(part 1 of 3)
# Autodesk Inventor assembly: DesignRootModel^PCB_ESP32-C3-MINI-1_V1(2)_PCB_ESP32-C3-MINI-1_V1
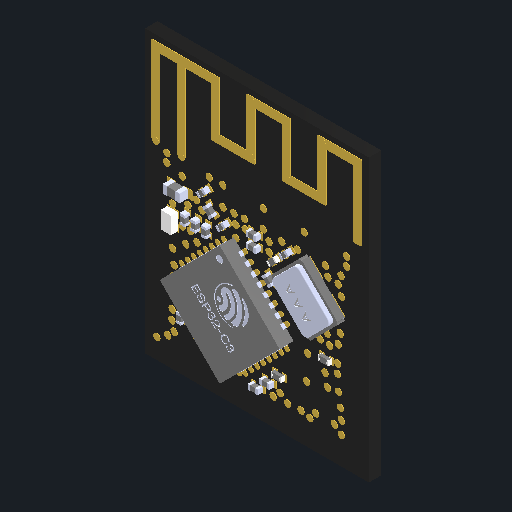
[picture p0: Inventor's stored thumbnail of the model, 512x512]
Saved by Autodesk Inventor 2026.1 (Build 301233000, 233)
## iProperties
Created: 2025-11-22
Part Number: DesignRootModel^PCB_ESP32-C3-MINI-1_V1(2)_PCB_ESP32-C3-MINI-1_V1
Document SubType Name: Assembly
Designer: micyg
Author: micyg
## Documents named in this file (333)
- C:\Users\micyg\Projects\virtual_pet\VirtualBlob\Mechanical\boards\MainBoard\MainBoard_0_4_0\VirtualBlob_MainBoard_0.4.0\VirtualBlob_MainBoard_0.4.0\DesignRootModel^PCB_ESP32-C3-MINI-1_V1(2)_PCB_ESP32-C3-MINI-1_.iam
- C:\Users\micyg\Projects\virtual_pet\VirtualBlob\Mechanical\boards\MainBoard\MainBoard_0_4_0\VirtualBlob_MainBoard_0.4.0\VirtualBlob_MainBoard_0.4.0\Submodel-SOD882_part^DesignRootModel_PCB_ESP32-C3-MINI-1_V1(2).iam
- C:\Users\micyg\Projects\virtual_pet\VirtualBlob\Mechanical\boards\MainBoard\MainBoard_0_4_0\VirtualBlob_MainBoard_0.4.0\VirtualBlob_MainBoard_0.4.0\Submodel-R0201_part^DesignRootModel_PCB_ESP32-C3-MINI-1_V1(2)_.iam
- C:\Users\micyg\Projects\virtual_pet\VirtualBlob\Mechanical\boards\MainBoard\MainBoard_0_4_0\VirtualBlob_MainBoard_0.4.0\VirtualBlob_MainBoard_0.4.0\Submodel-MINI-ANT-TYPED-H_1968823293_part^DesignRootModel_PCB_.iam
- C:\Users\micyg\Projects\virtual_pet\VirtualBlob\Mechanical\boards\MainBoard\MainBoard_0_4_0\VirtualBlob_MainBoard_0.4.0\VirtualBlob_MainBoard_0.4.0\Submodel-C0402_part^DesignRootModel_PCB_ESP32-C3-MINI-1_V1(2)_.iam
- C:\Users\micyg\Projects\virtual_pet\VirtualBlob\Mechanical\boards\MainBoard\MainBoard_0_4_0\VirtualBlob_MainBoard_0.4.0\VirtualBlob_MainBoard_0.4.0\Submodel-R0201_part^DesignRootModel_PCB_ESP32-C3-MINI-1_V1(2)__1.iam
- C:\Users\micyg\Projects\virtual_pet\VirtualBlob\Mechanical\boards\MainBoard\MainBoard_0_4_0\VirtualBlob_MainBoard_0.4.0\VirtualBlob_MainBoard_0.4.0\Submodel-C0201_part^DesignRootModel_PCB_ESP32-C3-MINI-1_V1(2)_.iam
- C:\Users\micyg\Projects\virtual_pet\VirtualBlob\Mechanical\boards\MainBoard\MainBoard_0_4_0\VirtualBlob_MainBoard_0.4.0\VirtualBlob_MainBoard_0.4.0\Submodel-R0201_part^DesignRootModel_PCB_ESP32-C3-MINI-1_V1(2)__2.iam
- C:\Users\micyg\Projects\virtual_pet\VirtualBlob\Mechanical\boards\MainBoard\MainBoard_0_4_0\VirtualBlob_MainBoard_0.4.0\VirtualBlob_MainBoard_0.4.0\Submodel-C0201_part^DesignRootModel_PCB_ESP32-C3-MINI-1_V1(2)__1.iam
- C:\Users\micyg\Projects\virtual_pet\VirtualBlob\Mechanical\boards\MainBoard\MainBoard_0_4_0\VirtualBlob_MainBoard_0.4.0\VirtualBlob_MainBoard_0.4.0\Submodel-C0201_part^DesignRootModel_PCB_ESP32-C3-MINI-1_V1(2)__2.iam
- C:\Users\micyg\Projects\virtual_pet\VirtualBlob\Mechanical\boards\MainBoard\MainBoard_0_4_0\VirtualBlob_MainBoard_0.4.0\VirtualBlob_MainBoard_0.4.0\Submodel-C0201_part^DesignRootModel_PCB_ESP32-C3-MINI-1_V1(2)__3.iam
- C:\Users\micyg\Projects\virtual_pet\VirtualBlob\Mechanical\boards\MainBoard\MainBoard_0_4_0\VirtualBlob_MainBoard_0.4.0\VirtualBlob_MainBoard_0.4.0\Submodel-C0201_part^DesignRootModel_PCB_ESP32-C3-MINI-1_V1(2)__4.iam
- C:\Users\micyg\Projects\virtual_pet\VirtualBlob\Mechanical\boards\MainBoard\MainBoard_0_4_0\VirtualBlob_MainBoard_0.4.0\VirtualBlob_MainBoard_0.4.0\Submodel-C0201_part^DesignRootModel_PCB_ESP32-C3-MINI-1_V1(2)__5.iam
- C:\Users\micyg\Projects\virtual_pet\VirtualBlob\Mechanical\boards\MainBoard\MainBoard_0_4_0\VirtualBlob_MainBoard_0.4.0\VirtualBlob_MainBoard_0.4.0\Submodel-C0201_part^DesignRootModel_PCB_ESP32-C3-MINI-1_V1(2)__6.iam
- C:\Users\micyg\Projects\virtual_pet\VirtualBlob\Mechanical\boards\MainBoard\MainBoard_0_4_0\VirtualBlob_MainBoard_0.4.0\VirtualBlob_MainBoard_0.4.0\Submodel-C0201_part^DesignRootModel_PCB_ESP32-C3-MINI-1_V1(2)__7.iam
- C:\Users\micyg\Projects\virtual_pet\VirtualBlob\Mechanical\boards\MainBoard\MainBoard_0_4_0\VirtualBlob_MainBoard_0.4.0\VirtualBlob_MainBoard_0.4.0\Submodel-C0201_part^DesignRootModel_PCB_ESP32-C3-MINI-1_V1(2)__8.iam
- C:\Users\micyg\Projects\virtual_pet\VirtualBlob\Mechanical\boards\MainBoard\MainBoard_0_4_0\VirtualBlob_MainBoard_0.4.0\VirtualBlob_MainBoard_0.4.0\Submodel-C0201_part^DesignRootModel_PCB_ESP32-C3-MINI-1_V1(2)__9.iam
- C:\Users\micyg\Projects\virtual_pet\VirtualBlob\Mechanical\boards\MainBoard\MainBoard_0_4_0\VirtualBlob_MainBoard_0.4.0\VirtualBlob_MainBoard_0.4.0\Submodel-L0201_part^DesignRootModel_PCB_ESP32-C3-MINI-1_V1(2)_.iam
- C:\Users\micyg\Projects\virtual_pet\VirtualBlob\Mechanical\boards\MainBoard\MainBoard_0_4_0\VirtualBlob_MainBoard_0.4.0\VirtualBlob_MainBoard_0.4.0\Submodel-L0201_part^DesignRootModel_PCB_ESP32-C3-MINI-1_V1(2)__1.iam
- C:\Users\micyg\Projects\virtual_pet\VirtualBlob\Mechanical\boards\MainBoard\MainBoard_0_4_0\VirtualBlob_MainBoard_0.4.0\VirtualBlob_MainBoard_0.4.0\Submodel-XTAL3225_part^DesignRootModel_PCB_ESP32-C3-MINI-1_V1(.iam
- C:\Users\micyg\Projects\virtual_pet\VirtualBlob\Mechanical\boards\MainBoard\MainBoard_0_4_0\VirtualBlob_MainBoard_0.4.0\VirtualBlob_MainBoard_0.4.0\Submodel-QFN32_0P5_5_part^DesignRootModel_PCB_ESP32-C3-MINI-1_.iam
- C:\Users\micyg\Projects\virtual_pet\VirtualBlob\Mechanical\boards\MainBoard\MainBoard_0_4_0\VirtualBlob_MainBoard_0.4.0\VirtualBlob_MainBoard_0.4.0\Submodel-C0201_part^DesignRootModel_PCB_ESP32-C3-MINI-1_V1(2)__10.iam
- C:\Users\micyg\Projects\virtual_pet\VirtualBlob\Mechanical\boards\MainBoard\MainBoard_0_4_0\VirtualBlob_MainBoard_0.4.0\VirtualBlob_MainBoard_0.4.0\uid__4^DesignRootModel_PCB_ESP32-C3-MINI-1_V1(2)_PCB_ESP32-C3-.ipt
- C:\Users\micyg\Projects\virtual_pet\VirtualBlob\Mechanical\boards\MainBoard\MainBoard_0_4_0\VirtualBlob_MainBoard_0.4.0\VirtualBlob_MainBoard_0.4.0\uid__4-22^DesignRootModel_PCB_ESP32-C3-MINI-1_V1(2)_PCB_ESP32-.ipt
- C:\Users\micyg\Projects\virtual_pet\VirtualBlob\Mechanical\boards\MainBoard\MainBoard_0_4_0\VirtualBlob_MainBoard_0.4.0\VirtualBlob_MainBoard_0.4.0\uid__4-23^DesignRootModel_PCB_ESP32-C3-MINI-1_V1(2)_PCB_ESP32-.ipt
- C:\Users\micyg\Projects\virtual_pet\VirtualBlob\Mechanical\boards\MainBoard\MainBoard_0_4_0\VirtualBlob_MainBoard_0.4.0\VirtualBlob_MainBoard_0.4.0\uid__4-24^DesignRootModel_PCB_ESP32-C3-MINI-1_V1(2)_PCB_ESP32-.ipt
- C:\Users\micyg\Projects\virtual_pet\VirtualBlob\Mechanical\boards\MainBoard\MainBoard_0_4_0\VirtualBlob_MainBoard_0.4.0\VirtualBlob_MainBoard_0.4.0\uid__4-25^DesignRootModel_PCB_ESP32-C3-MINI-1_V1(2)_PCB_ESP32-.ipt
- C:\Users\micyg\Projects\virtual_pet\VirtualBlob\Mechanical\boards\MainBoard\MainBoard_0_4_0\VirtualBlob_MainBoard_0.4.0\VirtualBlob_MainBoard_0.4.0\uid__4-26^DesignRootModel_PCB_ESP32-C3-MINI-1_V1(2)_PCB_ESP32-.ipt
- C:\Users\micyg\Projects\virtual_pet\VirtualBlob\Mechanical\boards\MainBoard\MainBoard_0_4_0\VirtualBlob_MainBoard_0.4.0\VirtualBlob_MainBoard_0.4.0\uid__4-27^DesignRootModel_PCB_ESP32-C3-MINI-1_V1(2)_PCB_ESP32-.ipt
- C:\Users\micyg\Projects\virtual_pet\VirtualBlob\Mechanical\boards\MainBoard\MainBoard_0_4_0\VirtualBlob_MainBoard_0.4.0\VirtualBlob_MainBoard_0.4.0\uid__4-28^DesignRootModel_PCB_ESP32-C3-MINI-1_V1(2)_PCB_ESP32-.ipt
- C:\Users\micyg\Projects\virtual_pet\VirtualBlob\Mechanical\boards\MainBoard\MainBoard_0_4_0\VirtualBlob_MainBoard_0.4.0\VirtualBlob_MainBoard_0.4.0\uid__4-29^DesignRootModel_PCB_ESP32-C3-MINI-1_V1(2)_PCB_ESP32-.ipt
- C:\Users\micyg\Projects\virtual_pet\VirtualBlob\Mechanical\boards\MainBoard\MainBoard_0_4_0\VirtualBlob_MainBoard_0.4.0\VirtualBlob_MainBoard_0.4.0\uid__4-30^DesignRootModel_PCB_ESP32-C3-MINI-1_V1(2)_PCB_ESP32-.ipt
- C:\Users\micyg\Projects\virtual_pet\VirtualBlob\Mechanical\boards\MainBoard\MainBoard_0_4_0\VirtualBlob_MainBoard_0.4.0\VirtualBlob_MainBoard_0.4.0\uid__4-31^DesignRootModel_PCB_ESP32-C3-MINI-1_V1(2)_PCB_ESP32-.ipt
- C:\Users\micyg\Projects\virtual_pet\VirtualBlob\Mechanical\boards\MainBoard\MainBoard_0_4_0\VirtualBlob_MainBoard_0.4.0\VirtualBlob_MainBoard_0.4.0\uid__4-32^DesignRootModel_PCB_ESP32-C3-MINI-1_V1(2)_PCB_ESP32-.ipt
- C:\Users\micyg\Projects\virtual_pet\VirtualBlob\Mechanical\boards\MainBoard\MainBoard_0_4_0\VirtualBlob_MainBoard_0.4.0\VirtualBlob_MainBoard_0.4.0\uid__4-33^DesignRootModel_PCB_ESP32-C3-MINI-1_V1(2)_PCB_ESP32-.ipt
- C:\Users\micyg\Projects\virtual_pet\VirtualBlob\Mechanical\boards\MainBoard\MainBoard_0_4_0\VirtualBlob_MainBoard_0.4.0\VirtualBlob_MainBoard_0.4.0\uid__4-34^DesignRootModel_PCB_ESP32-C3-MINI-1_V1(2)_PCB_ESP32-.ipt
- C:\Users\micyg\Projects\virtual_pet\VirtualBlob\Mechanical\boards\MainBoard\MainBoard_0_4_0\VirtualBlob_MainBoard_0.4.0\VirtualBlob_MainBoard_0.4.0\uid__4-35^DesignRootModel_PCB_ESP32-C3-MINI-1_V1(2)_PCB_ESP32-.ipt
- C:\Users\micyg\Projects\virtual_pet\VirtualBlob\Mechanical\boards\MainBoard\MainBoard_0_4_0\VirtualBlob_MainBoard_0.4.0\VirtualBlob_MainBoard_0.4.0\uid__4-36^DesignRootModel_PCB_ESP32-C3-MINI-1_V1(2)_PCB_ESP32-.ipt
- C:\Users\micyg\Projects\virtual_pet\VirtualBlob\Mechanical\boards\MainBoard\MainBoard_0_4_0\VirtualBlob_MainBoard_0.4.0\VirtualBlob_MainBoard_0.4.0\uid__4-37^DesignRootModel_PCB_ESP32-C3-MINI-1_V1(2)_PCB_ESP32-.ipt
- C:\Users\micyg\Projects\virtual_pet\VirtualBlob\Mechanical\boards\MainBoard\MainBoard_0_4_0\VirtualBlob_MainBoard_0.4.0\VirtualBlob_MainBoard_0.4.0\uid__4-38^DesignRootModel_PCB_ESP32-C3-MINI-1_V1(2)_PCB_ESP32-.ipt
- C:\Users\micyg\Projects\virtual_pet\VirtualBlob\Mechanical\boards\MainBoard\MainBoard_0_4_0\VirtualBlob_MainBoard_0.4.0\VirtualBlob_MainBoard_0.4.0\uid__4-39^DesignRootModel_PCB_ESP32-C3-MINI-1_V1(2)_PCB_ESP32-.ipt
- C:\Users\micyg\Projects\virtual_pet\VirtualBlob\Mechanical\boards\MainBoard\MainBoard_0_4_0\VirtualBlob_MainBoard_0.4.0\VirtualBlob_MainBoard_0.4.0\uid__4-40^DesignRootModel_PCB_ESP32-C3-MINI-1_V1(2)_PCB_ESP32-.ipt
- C:\Users\micyg\Projects\virtual_pet\VirtualBlob\Mechanical\boards\MainBoard\MainBoard_0_4_0\VirtualBlob_MainBoard_0.4.0\VirtualBlob_MainBoard_0.4.0\uid__4-41^DesignRootModel_PCB_ESP32-C3-MINI-1_V1(2)_PCB_ESP32-.ipt
- C:\Users\micyg\Projects\virtual_pet\VirtualBlob\Mechanical\boards\MainBoard\MainBoard_0_4_0\VirtualBlob_MainBoard_0.4.0\VirtualBlob_MainBoard_0.4.0\uid__4-42^DesignRootModel_PCB_ESP32-C3-MINI-1_V1(2)_PCB_ESP32-.ipt
- C:\Users\micyg\Projects\virtual_pet\VirtualBlob\Mechanical\boards\MainBoard\MainBoard_0_4_0\VirtualBlob_MainBoard_0.4.0\VirtualBlob_MainBoard_0.4.0\uid__4-43^DesignRootModel_PCB_ESP32-C3-MINI-1_V1(2)_PCB_ESP32-.ipt
- C:\Users\micyg\Projects\virtual_pet\VirtualBlob\Mechanical\boards\MainBoard\MainBoard_0_4_0\VirtualBlob_MainBoard_0.4.0\VirtualBlob_MainBoard_0.4.0\uid__4-44^DesignRootModel_PCB_ESP32-C3-MINI-1_V1(2)_PCB_ESP32-.ipt
- C:\Users\micyg\Projects\virtual_pet\VirtualBlob\Mechanical\boards\MainBoard\MainBoard_0_4_0\VirtualBlob_MainBoard_0.4.0\VirtualBlob_MainBoard_0.4.0\uid__4-45^DesignRootModel_PCB_ESP32-C3-MINI-1_V1(2)_PCB_ESP32-.ipt
- C:\Users\micyg\Projects\virtual_pet\VirtualBlob\Mechanical\boards\MainBoard\MainBoard_0_4_0\VirtualBlob_MainBoard_0.4.0\VirtualBlob_MainBoard_0.4.0\uid__4-46^DesignRootModel_PCB_ESP32-C3-MINI-1_V1(2)_PCB_ESP32-.ipt
- C:\Users\micyg\Projects\virtual_pet\VirtualBlob\Mechanical\boards\MainBoard\MainBoard_0_4_0\VirtualBlob_MainBoard_0.4.0\VirtualBlob_MainBoard_0.4.0\uid__4-47^DesignRootModel_PCB_ESP32-C3-MINI-1_V1(2)_PCB_ESP32-.ipt
- C:\Users\micyg\Projects\virtual_pet\VirtualBlob\Mechanical\boards\MainBoard\MainBoard_0_4_0\VirtualBlob_MainBoard_0.4.0\VirtualBlob_MainBoard_0.4.0\uid__4-48^DesignRootModel_PCB_ESP32-C3-MINI-1_V1(2)_PCB_ESP32-.ipt
- C:\Users\micyg\Projects\virtual_pet\VirtualBlob\Mechanical\boards\MainBoard\MainBoard_0_4_0\VirtualBlob_MainBoard_0.4.0\VirtualBlob_MainBoard_0.4.0\uid__4-49^DesignRootModel_PCB_ESP32-C3-MINI-1_V1(2)_PCB_ESP32-.ipt
- C:\Users\micyg\Projects\virtual_pet\VirtualBlob\Mechanical\boards\MainBoard\MainBoard_0_4_0\VirtualBlob_MainBoard_0.4.0\VirtualBlob_MainBoard_0.4.0\uid__4-50^DesignRootModel_PCB_ESP32-C3-MINI-1_V1(2)_PCB_ESP32-.ipt
- C:\Users\micyg\Projects\virtual_pet\VirtualBlob\Mechanical\boards\MainBoard\MainBoard_0_4_0\VirtualBlob_MainBoard_0.4.0\VirtualBlob_MainBoard_0.4.0\uid__4-51^DesignRootModel_PCB_ESP32-C3-MINI-1_V1(2)_PCB_ESP32-.ipt
- C:\Users\micyg\Projects\virtual_pet\VirtualBlob\Mechanical\boards\MainBoard\MainBoard_0_4_0\VirtualBlob_MainBoard_0.4.0\VirtualBlob_MainBoard_0.4.0\uid__4-52^DesignRootModel_PCB_ESP32-C3-MINI-1_V1(2)_PCB_ESP32-.ipt
- C:\Users\micyg\Projects\virtual_pet\VirtualBlob\Mechanical\boards\MainBoard\MainBoard_0_4_0\VirtualBlob_MainBoard_0.4.0\VirtualBlob_MainBoard_0.4.0\uid__4-53^DesignRootModel_PCB_ESP32-C3-MINI-1_V1(2)_PCB_ESP32-.ipt
- C:\Users\micyg\Projects\virtual_pet\VirtualBlob\Mechanical\boards\MainBoard\MainBoard_0_4_0\VirtualBlob_MainBoard_0.4.0\VirtualBlob_MainBoard_0.4.0\uid__4-54^DesignRootModel_PCB_ESP32-C3-MINI-1_V1(2)_PCB_ESP32-.ipt
- C:\Users\micyg\Projects\virtual_pet\VirtualBlob\Mechanical\boards\MainBoard\MainBoard_0_4_0\VirtualBlob_MainBoard_0.4.0\VirtualBlob_MainBoard_0.4.0\uid__4-55^DesignRootModel_PCB_ESP32-C3-MINI-1_V1(2)_PCB_ESP32-.ipt
- C:\Users\micyg\Projects\virtual_pet\VirtualBlob\Mechanical\boards\MainBoard\MainBoard_0_4_0\VirtualBlob_MainBoard_0.4.0\VirtualBlob_MainBoard_0.4.0\uid__4-56^DesignRootModel_PCB_ESP32-C3-MINI-1_V1(2)_PCB_ESP32-.ipt
- C:\Users\micyg\Projects\virtual_pet\VirtualBlob\Mechanical\boards\MainBoard\MainBoard_0_4_0\VirtualBlob_MainBoard_0.4.0\VirtualBlob_MainBoard_0.4.0\uid__4-57^DesignRootModel_PCB_ESP32-C3-MINI-1_V1(2)_PCB_ESP32-.ipt
- C:\Users\micyg\Projects\virtual_pet\VirtualBlob\Mechanical\boards\MainBoard\MainBoard_0_4_0\VirtualBlob_MainBoard_0.4.0\VirtualBlob_MainBoard_0.4.0\uid__4-58^DesignRootModel_PCB_ESP32-C3-MINI-1_V1(2)_PCB_ESP32-.ipt
- C:\Users\micyg\Projects\virtual_pet\VirtualBlob\Mechanical\boards\MainBoard\MainBoard_0_4_0\VirtualBlob_MainBoard_0.4.0\VirtualBlob_MainBoard_0.4.0\uid__4-59^DesignRootModel_PCB_ESP32-C3-MINI-1_V1(2)_PCB_ESP32-.ipt
- C:\Users\micyg\Projects\virtual_pet\VirtualBlob\Mechanical\boards\MainBoard\MainBoard_0_4_0\VirtualBlob_MainBoard_0.4.0\VirtualBlob_MainBoard_0.4.0\uid__4-60^DesignRootModel_PCB_ESP32-C3-MINI-1_V1(2)_PCB_ESP32-.ipt
- C:\Users\micyg\Projects\virtual_pet\VirtualBlob\Mechanical\boards\MainBoard\MainBoard_0_4_0\VirtualBlob_MainBoard_0.4.0\VirtualBlob_MainBoard_0.4.0\uid__4-61^DesignRootModel_PCB_ESP32-C3-MINI-1_V1(2)_PCB_ESP32-.ipt
- C:\Users\micyg\Projects\virtual_pet\VirtualBlob\Mechanical\boards\MainBoard\MainBoard_0_4_0\VirtualBlob_MainBoard_0.4.0\VirtualBlob_MainBoard_0.4.0\uid__4-62^DesignRootModel_PCB_ESP32-C3-MINI-1_V1(2)_PCB_ESP32-.ipt
- C:\Users\micyg\Projects\virtual_pet\VirtualBlob\Mechanical\boards\MainBoard\MainBoard_0_4_0\VirtualBlob_MainBoard_0.4.0\VirtualBlob_MainBoard_0.4.0\uid__4-63^DesignRootModel_PCB_ESP32-C3-MINI-1_V1(2)_PCB_ESP32-.ipt
- C:\Users\micyg\Projects\virtual_pet\VirtualBlob\Mechanical\boards\MainBoard\MainBoard_0_4_0\VirtualBlob_MainBoard_0.4.0\VirtualBlob_MainBoard_0.4.0\uid__4-64^DesignRootModel_PCB_ESP32-C3-MINI-1_V1(2)_PCB_ESP32-.ipt
- C:\Users\micyg\Projects\virtual_pet\VirtualBlob\Mechanical\boards\MainBoard\MainBoard_0_4_0\VirtualBlob_MainBoard_0.4.0\VirtualBlob_MainBoard_0.4.0\uid__4-65^DesignRootModel_PCB_ESP32-C3-MINI-1_V1(2)_PCB_ESP32-.ipt
- C:\Users\micyg\Projects\virtual_pet\VirtualBlob\Mechanical\boards\MainBoard\MainBoard_0_4_0\VirtualBlob_MainBoard_0.4.0\VirtualBlob_MainBoard_0.4.0\uid__4-66^DesignRootModel_PCB_ESP32-C3-MINI-1_V1(2)_PCB_ESP32-.ipt
- C:\Users\micyg\Projects\virtual_pet\VirtualBlob\Mechanical\boards\MainBoard\MainBoard_0_4_0\VirtualBlob_MainBoard_0.4.0\VirtualBlob_MainBoard_0.4.0\uid__4-67^DesignRootModel_PCB_ESP32-C3-MINI-1_V1(2)_PCB_ESP32-.ipt
- C:\Users\micyg\Projects\virtual_pet\VirtualBlob\Mechanical\boards\MainBoard\MainBoard_0_4_0\VirtualBlob_MainBoard_0.4.0\VirtualBlob_MainBoard_0.4.0\uid__4-68^DesignRootModel_PCB_ESP32-C3-MINI-1_V1(2)_PCB_ESP32-.ipt
- C:\Users\micyg\Projects\virtual_pet\VirtualBlob\Mechanical\boards\MainBoard\MainBoard_0_4_0\VirtualBlob_MainBoard_0.4.0\VirtualBlob_MainBoard_0.4.0\uid__4-69^DesignRootModel_PCB_ESP32-C3-MINI-1_V1(2)_PCB_ESP32-.ipt
- C:\Users\micyg\Projects\virtual_pet\VirtualBlob\Mechanical\boards\MainBoard\MainBoard_0_4_0\VirtualBlob_MainBoard_0.4.0\VirtualBlob_MainBoard_0.4.0\uid__4-70^DesignRootModel_PCB_ESP32-C3-MINI-1_V1(2)_PCB_ESP32-.ipt
- C:\Users\micyg\Projects\virtual_pet\VirtualBlob\Mechanical\boards\MainBoard\MainBoard_0_4_0\VirtualBlob_MainBoard_0.4.0\VirtualBlob_MainBoard_0.4.0\uid__4-71^DesignRootModel_PCB_ESP32-C3-MINI-1_V1(2)_PCB_ESP32-.ipt
- C:\Users\micyg\Projects\virtual_pet\VirtualBlob\Mechanical\boards\MainBoard\MainBoard_0_4_0\VirtualBlob_MainBoard_0.4.0\VirtualBlob_MainBoard_0.4.0\uid__4-72^DesignRootModel_PCB_ESP32-C3-MINI-1_V1(2)_PCB_ESP32-.ipt
- C:\Users\micyg\Projects\virtual_pet\VirtualBlob\Mechanical\boards\MainBoard\MainBoard_0_4_0\VirtualBlob_MainBoard_0.4.0\VirtualBlob_MainBoard_0.4.0\uid__4-73^DesignRootModel_PCB_ESP32-C3-MINI-1_V1(2)_PCB_ESP32-.ipt
- C:\Users\micyg\Projects\virtual_pet\VirtualBlob\Mechanical\boards\MainBoard\MainBoard_0_4_0\VirtualBlob_MainBoard_0.4.0\VirtualBlob_MainBoard_0.4.0\uid__4-74^DesignRootModel_PCB_ESP32-C3-MINI-1_V1(2)_PCB_ESP32-.ipt
- C:\Users\micyg\Projects\virtual_pet\VirtualBlob\Mechanical\boards\MainBoard\MainBoard_0_4_0\VirtualBlob_MainBoard_0.4.0\VirtualBlob_MainBoard_0.4.0\uid__4-75^DesignRootModel_PCB_ESP32-C3-MINI-1_V1(2)_PCB_ESP32-.ipt
- C:\Users\micyg\Projects\virtual_pet\VirtualBlob\Mechanical\boards\MainBoard\MainBoard_0_4_0\VirtualBlob_MainBoard_0.4.0\VirtualBlob_MainBoard_0.4.0\uid__4-76^DesignRootModel_PCB_ESP32-C3-MINI-1_V1(2)_PCB_ESP32-.ipt
- C:\Users\micyg\Projects\virtual_pet\VirtualBlob\Mechanical\boards\MainBoard\MainBoard_0_4_0\VirtualBlob_MainBoard_0.4.0\VirtualBlob_MainBoard_0.4.0\uid__4-77^DesignRootModel_PCB_ESP32-C3-MINI-1_V1(2)_PCB_ESP32-.ipt
- C:\Users\micyg\Projects\virtual_pet\VirtualBlob\Mechanical\boards\MainBoard\MainBoard_0_4_0\VirtualBlob_MainBoard_0.4.0\VirtualBlob_MainBoard_0.4.0\uid__4-78^DesignRootModel_PCB_ESP32-C3-MINI-1_V1(2)_PCB_ESP32-.ipt
- C:\Users\micyg\Projects\virtual_pet\VirtualBlob\Mechanical\boards\MainBoard\MainBoard_0_4_0\VirtualBlob_MainBoard_0.4.0\VirtualBlob_MainBoard_0.4.0\uid__4-79^DesignRootModel_PCB_ESP32-C3-MINI-1_V1(2)_PCB_ESP32-.ipt
- C:\Users\micyg\Projects\virtual_pet\VirtualBlob\Mechanical\boards\MainBoard\MainBoard_0_4_0\VirtualBlob_MainBoard_0.4.0\VirtualBlob_MainBoard_0.4.0\uid__4-80^DesignRootModel_PCB_ESP32-C3-MINI-1_V1(2)_PCB_ESP32-.ipt
- C:\Users\micyg\Projects\virtual_pet\VirtualBlob\Mechanical\boards\MainBoard\MainBoard_0_4_0\VirtualBlob_MainBoard_0.4.0\VirtualBlob_MainBoard_0.4.0\uid__4-81^DesignRootModel_PCB_ESP32-C3-MINI-1_V1(2)_PCB_ESP32-.ipt
- C:\Users\micyg\Projects\virtual_pet\VirtualBlob\Mechanical\boards\MainBoard\MainBoard_0_4_0\VirtualBlob_MainBoard_0.4.0\VirtualBlob_MainBoard_0.4.0\uid__4-82^DesignRootModel_PCB_ESP32-C3-MINI-1_V1(2)_PCB_ESP32-.ipt
- C:\Users\micyg\Projects\virtual_pet\VirtualBlob\Mechanical\boards\MainBoard\MainBoard_0_4_0\VirtualBlob_MainBoard_0.4.0\VirtualBlob_MainBoard_0.4.0\uid__4-83^DesignRootModel_PCB_ESP32-C3-MINI-1_V1(2)_PCB_ESP32-.ipt
- C:\Users\micyg\Projects\virtual_pet\VirtualBlob\Mechanical\boards\MainBoard\MainBoard_0_4_0\VirtualBlob_MainBoard_0.4.0\VirtualBlob_MainBoard_0.4.0\uid__4-84^DesignRootModel_PCB_ESP32-C3-MINI-1_V1(2)_PCB_ESP32-.ipt
- C:\Users\micyg\Projects\virtual_pet\VirtualBlob\Mechanical\boards\MainBoard\MainBoard_0_4_0\VirtualBlob_MainBoard_0.4.0\VirtualBlob_MainBoard_0.4.0\uid__4-85^DesignRootModel_PCB_ESP32-C3-MINI-1_V1(2)_PCB_ESP32-.ipt
- C:\Users\micyg\Projects\virtual_pet\VirtualBlob\Mechanical\boards\MainBoard\MainBoard_0_4_0\VirtualBlob_MainBoard_0.4.0\VirtualBlob_MainBoard_0.4.0\uid__4-86^DesignRootModel_PCB_ESP32-C3-MINI-1_V1(2)_PCB_ESP32-.ipt
- C:\Users\micyg\Projects\virtual_pet\VirtualBlob\Mechanical\boards\MainBoard\MainBoard_0_4_0\VirtualBlob_MainBoard_0.4.0\VirtualBlob_MainBoard_0.4.0\uid__4-87^DesignRootModel_PCB_ESP32-C3-MINI-1_V1(2)_PCB_ESP32-.ipt
- C:\Users\micyg\Projects\virtual_pet\VirtualBlob\Mechanical\boards\MainBoard\MainBoard_0_4_0\VirtualBlob_MainBoard_0.4.0\VirtualBlob_MainBoard_0.4.0\uid__4-88^DesignRootModel_PCB_ESP32-C3-MINI-1_V1(2)_PCB_ESP32-.ipt
- C:\Users\micyg\Projects\virtual_pet\VirtualBlob\Mechanical\boards\MainBoard\MainBoard_0_4_0\VirtualBlob_MainBoard_0.4.0\VirtualBlob_MainBoard_0.4.0\uid__4-89^DesignRootModel_PCB_ESP32-C3-MINI-1_V1(2)_PCB_ESP32-.ipt
- C:\Users\micyg\Projects\virtual_pet\VirtualBlob\Mechanical\boards\MainBoard\MainBoard_0_4_0\VirtualBlob_MainBoard_0.4.0\VirtualBlob_MainBoard_0.4.0\uid__4-90^DesignRootModel_PCB_ESP32-C3-MINI-1_V1(2)_PCB_ESP32-.ipt
- C:\Users\micyg\Projects\virtual_pet\VirtualBlob\Mechanical\boards\MainBoard\MainBoard_0_4_0\VirtualBlob_MainBoard_0.4.0\VirtualBlob_MainBoard_0.4.0\uid__4-91^DesignRootModel_PCB_ESP32-C3-MINI-1_V1(2)_PCB_ESP32-.ipt
- C:\Users\micyg\Projects\virtual_pet\VirtualBlob\Mechanical\boards\MainBoard\MainBoard_0_4_0\VirtualBlob_MainBoard_0.4.0\VirtualBlob_MainBoard_0.4.0\uid__4-92^DesignRootModel_PCB_ESP32-C3-MINI-1_V1(2)_PCB_ESP32-.ipt
- C:\Users\micyg\Projects\virtual_pet\VirtualBlob\Mechanical\boards\MainBoard\MainBoard_0_4_0\VirtualBlob_MainBoard_0.4.0\VirtualBlob_MainBoard_0.4.0\uid__4-93^DesignRootModel_PCB_ESP32-C3-MINI-1_V1(2)_PCB_ESP32-.ipt
- C:\Users\micyg\Projects\virtual_pet\VirtualBlob\Mechanical\boards\MainBoard\MainBoard_0_4_0\VirtualBlob_MainBoard_0.4.0\VirtualBlob_MainBoard_0.4.0\uid__4-94^DesignRootModel_PCB_ESP32-C3-MINI-1_V1(2)_PCB_ESP32-.ipt
- C:\Users\micyg\Projects\virtual_pet\VirtualBlob\Mechanical\boards\MainBoard\MainBoard_0_4_0\VirtualBlob_MainBoard_0.4.0\VirtualBlob_MainBoard_0.4.0\uid__4-95^DesignRootModel_PCB_ESP32-C3-MINI-1_V1(2)_PCB_ESP32-.ipt
- C:\Users\micyg\Projects\virtual_pet\VirtualBlob\Mechanical\boards\MainBoard\MainBoard_0_4_0\VirtualBlob_MainBoard_0.4.0\VirtualBlob_MainBoard_0.4.0\uid__4-96^DesignRootModel_PCB_ESP32-C3-MINI-1_V1(2)_PCB_ESP32-.ipt
- C:\Users\micyg\Projects\virtual_pet\VirtualBlob\Mechanical\boards\MainBoard\MainBoard_0_4_0\VirtualBlob_MainBoard_0.4.0\VirtualBlob_MainBoard_0.4.0\uid__4-97^DesignRootModel_PCB_ESP32-C3-MINI-1_V1(2)_PCB_ESP32-.ipt
- C:\Users\micyg\Projects\virtual_pet\VirtualBlob\Mechanical\boards\MainBoard\MainBoard_0_4_0\VirtualBlob_MainBoard_0.4.0\VirtualBlob_MainBoard_0.4.0\uid__4-98^DesignRootModel_PCB_ESP32-C3-MINI-1_V1(2)_PCB_ESP32-.ipt
- C:\Users\micyg\Projects\virtual_pet\VirtualBlob\Mechanical\boards\MainBoard\MainBoard_0_4_0\VirtualBlob_MainBoard_0.4.0\VirtualBlob_MainBoard_0.4.0\uid__4-99^DesignRootModel_PCB_ESP32-C3-MINI-1_V1(2)_PCB_ESP32-.ipt
- C:\Users\micyg\Projects\virtual_pet\VirtualBlob\Mechanical\boards\MainBoard\MainBoard_0_4_0\VirtualBlob_MainBoard_0.4.0\VirtualBlob_MainBoard_0.4.0\uid__4-100^DesignRootModel_PCB_ESP32-C3-MINI-1_V1(2)_PCB_ESP32.ipt
- C:\Users\micyg\Projects\virtual_pet\VirtualBlob\Mechanical\boards\MainBoard\MainBoard_0_4_0\VirtualBlob_MainBoard_0.4.0\VirtualBlob_MainBoard_0.4.0\uid__4-101^DesignRootModel_PCB_ESP32-C3-MINI-1_V1(2)_PCB_ESP32.ipt
- C:\Users\micyg\Projects\virtual_pet\VirtualBlob\Mechanical\boards\MainBoard\MainBoard_0_4_0\VirtualBlob_MainBoard_0.4.0\VirtualBlob_MainBoard_0.4.0\uid__4-102^DesignRootModel_PCB_ESP32-C3-MINI-1_V1(2)_PCB_ESP32.ipt
- C:\Users\micyg\Projects\virtual_pet\VirtualBlob\Mechanical\boards\MainBoard\MainBoard_0_4_0\VirtualBlob_MainBoard_0.4.0\VirtualBlob_MainBoard_0.4.0\uid__4-103^DesignRootModel_PCB_ESP32-C3-MINI-1_V1(2)_PCB_ESP32.ipt
- C:\Users\micyg\Projects\virtual_pet\VirtualBlob\Mechanical\boards\MainBoard\MainBoard_0_4_0\VirtualBlob_MainBoard_0.4.0\VirtualBlob_MainBoard_0.4.0\uid__4-104^DesignRootModel_PCB_ESP32-C3-MINI-1_V1(2)_PCB_ESP32.ipt
- C:\Users\micyg\Projects\virtual_pet\VirtualBlob\Mechanical\boards\MainBoard\MainBoard_0_4_0\VirtualBlob_MainBoard_0.4.0\VirtualBlob_MainBoard_0.4.0\uid__4-105^DesignRootModel_PCB_ESP32-C3-MINI-1_V1(2)_PCB_ESP32.ipt
- C:\Users\micyg\Projects\virtual_pet\VirtualBlob\Mechanical\boards\MainBoard\MainBoard_0_4_0\VirtualBlob_MainBoard_0.4.0\VirtualBlob_MainBoard_0.4.0\uid__4-106^DesignRootModel_PCB_ESP32-C3-MINI-1_V1(2)_PCB_ESP32.ipt
- C:\Users\micyg\Projects\virtual_pet\VirtualBlob\Mechanical\boards\MainBoard\MainBoard_0_4_0\VirtualBlob_MainBoard_0.4.0\VirtualBlob_MainBoard_0.4.0\uid__4-107^DesignRootModel_PCB_ESP32-C3-MINI-1_V1(2)_PCB_ESP32.ipt
- C:\Users\micyg\Projects\virtual_pet\VirtualBlob\Mechanical\boards\MainBoard\MainBoard_0_4_0\VirtualBlob_MainBoard_0.4.0\VirtualBlob_MainBoard_0.4.0\uid__4-108^DesignRootModel_PCB_ESP32-C3-MINI-1_V1(2)_PCB_ESP32.ipt
- C:\Users\micyg\Projects\virtual_pet\VirtualBlob\Mechanical\boards\MainBoard\MainBoard_0_4_0\VirtualBlob_MainBoard_0.4.0\VirtualBlob_MainBoard_0.4.0\uid__4-109^DesignRootModel_PCB_ESP32-C3-MINI-1_V1(2)_PCB_ESP32.ipt
- C:\Users\micyg\Projects\virtual_pet\VirtualBlob\Mechanical\boards\MainBoard\MainBoard_0_4_0\VirtualBlob_MainBoard_0.4.0\VirtualBlob_MainBoard_0.4.0\uid__4-110^DesignRootModel_PCB_ESP32-C3-MINI-1_V1(2)_PCB_ESP32.ipt
- C:\Users\micyg\Projects\virtual_pet\VirtualBlob\Mechanical\boards\MainBoard\MainBoard_0_4_0\VirtualBlob_MainBoard_0.4.0\VirtualBlob_MainBoard_0.4.0\uid__4-111^DesignRootModel_PCB_ESP32-C3-MINI-1_V1(2)_PCB_ESP32.ipt
- C:\Users\micyg\Projects\virtual_pet\VirtualBlob\Mechanical\boards\MainBoard\MainBoard_0_4_0\VirtualBlob_MainBoard_0.4.0\VirtualBlob_MainBoard_0.4.0\uid__4-112^DesignRootModel_PCB_ESP32-C3-MINI-1_V1(2)_PCB_ESP32.ipt
- C:\Users\micyg\Projects\virtual_pet\VirtualBlob\Mechanical\boards\MainBoard\MainBoard_0_4_0\VirtualBlob_MainBoard_0.4.0\VirtualBlob_MainBoard_0.4.0\uid__4-113^DesignRootModel_PCB_ESP32-C3-MINI-1_V1(2)_PCB_ESP32.ipt
- C:\Users\micyg\Projects\virtual_pet\VirtualBlob\Mechanical\boards\MainBoard\MainBoard_0_4_0\VirtualBlob_MainBoard_0.4.0\VirtualBlob_MainBoard_0.4.0\uid__4-114^DesignRootModel_PCB_ESP32-C3-MINI-1_V1(2)_PCB_ESP32.ipt
- C:\Users\micyg\Projects\virtual_pet\VirtualBlob\Mechanical\boards\MainBoard\MainBoard_0_4_0\VirtualBlob_MainBoard_0.4.0\VirtualBlob_MainBoard_0.4.0\uid__4-115^DesignRootModel_PCB_ESP32-C3-MINI-1_V1(2)_PCB_ESP32.ipt
- C:\Users\micyg\Projects\virtual_pet\VirtualBlob\Mechanical\boards\MainBoard\MainBoard_0_4_0\VirtualBlob_MainBoard_0.4.0\VirtualBlob_MainBoard_0.4.0\uid__4-116^DesignRootModel_PCB_ESP32-C3-MINI-1_V1(2)_PCB_ESP32.ipt
- C:\Users\micyg\Projects\virtual_pet\VirtualBlob\Mechanical\boards\MainBoard\MainBoard_0_4_0\VirtualBlob_MainBoard_0.4.0\VirtualBlob_MainBoard_0.4.0\uid__4-117^DesignRootModel_PCB_ESP32-C3-MINI-1_V1(2)_PCB_ESP32.ipt
- C:\Users\micyg\Projects\virtual_pet\VirtualBlob\Mechanical\boards\MainBoard\MainBoard_0_4_0\VirtualBlob_MainBoard_0.4.0\VirtualBlob_MainBoard_0.4.0\uid__4-118^DesignRootModel_PCB_ESP32-C3-MINI-1_V1(2)_PCB_ESP32.ipt
- C:\Users\micyg\Projects\virtual_pet\VirtualBlob\Mechanical\boards\MainBoard\MainBoard_0_4_0\VirtualBlob_MainBoard_0.4.0\VirtualBlob_MainBoard_0.4.0\uid__4-119^DesignRootModel_PCB_ESP32-C3-MINI-1_V1(2)_PCB_ESP32.ipt
- C:\Users\micyg\Projects\virtual_pet\VirtualBlob\Mechanical\boards\MainBoard\MainBoard_0_4_0\VirtualBlob_MainBoard_0.4.0\VirtualBlob_MainBoard_0.4.0\uid__4-120^DesignRootModel_PCB_ESP32-C3-MINI-1_V1(2)_PCB_ESP32.ipt
- C:\Users\micyg\Projects\virtual_pet\VirtualBlob\Mechanical\boards\MainBoard\MainBoard_0_4_0\VirtualBlob_MainBoard_0.4.0\VirtualBlob_MainBoard_0.4.0\uid__4-121^DesignRootModel_PCB_ESP32-C3-MINI-1_V1(2)_PCB_ESP32.ipt
- C:\Users\micyg\Projects\virtual_pet\VirtualBlob\Mechanical\boards\MainBoard\MainBoard_0_4_0\VirtualBlob_MainBoard_0.4.0\VirtualBlob_MainBoard_0.4.0\uid__4-122^DesignRootModel_PCB_ESP32-C3-MINI-1_V1(2)_PCB_ESP32.ipt
- C:\Users\micyg\Projects\virtual_pet\VirtualBlob\Mechanical\boards\MainBoard\MainBoard_0_4_0\VirtualBlob_MainBoard_0.4.0\VirtualBlob_MainBoard_0.4.0\uid__4-123^DesignRootModel_PCB_ESP32-C3-MINI-1_V1(2)_PCB_ESP32.ipt
- C:\Users\micyg\Projects\virtual_pet\VirtualBlob\Mechanical\boards\MainBoard\MainBoard_0_4_0\VirtualBlob_MainBoard_0.4.0\VirtualBlob_MainBoard_0.4.0\uid__4-124^DesignRootModel_PCB_ESP32-C3-MINI-1_V1(2)_PCB_ESP32.ipt
- C:\Users\micyg\Projects\virtual_pet\VirtualBlob\Mechanical\boards\MainBoard\MainBoard_0_4_0\VirtualBlob_MainBoard_0.4.0\VirtualBlob_MainBoard_0.4.0\uid__4-125^DesignRootModel_PCB_ESP32-C3-MINI-1_V1(2)_PCB_ESP32.ipt
- C:\Users\micyg\Projects\virtual_pet\VirtualBlob\Mechanical\boards\MainBoard\MainBoard_0_4_0\VirtualBlob_MainBoard_0.4.0\VirtualBlob_MainBoard_0.4.0\uid__4-126^DesignRootModel_PCB_ESP32-C3-MINI-1_V1(2)_PCB_ESP32.ipt
- C:\Users\micyg\Projects\virtual_pet\VirtualBlob\Mechanical\boards\MainBoard\MainBoard_0_4_0\VirtualBlob_MainBoard_0.4.0\VirtualBlob_MainBoard_0.4.0\uid__4-127^DesignRootModel_PCB_ESP32-C3-MINI-1_V1(2)_PCB_ESP32.ipt
- C:\Users\micyg\Projects\virtual_pet\VirtualBlob\Mechanical\boards\MainBoard\MainBoard_0_4_0\VirtualBlob_MainBoard_0.4.0\VirtualBlob_MainBoard_0.4.0\uid__4-128^DesignRootModel_PCB_ESP32-C3-MINI-1_V1(2)_PCB_ESP32.ipt
- C:\Users\micyg\Projects\virtual_pet\VirtualBlob\Mechanical\boards\MainBoard\MainBoard_0_4_0\VirtualBlob_MainBoard_0.4.0\VirtualBlob_MainBoard_0.4.0\uid__4-129^DesignRootModel_PCB_ESP32-C3-MINI-1_V1(2)_PCB_ESP32.ipt
- C:\Users\micyg\Projects\virtual_pet\VirtualBlob\Mechanical\boards\MainBoard\MainBoard_0_4_0\VirtualBlob_MainBoard_0.4.0\VirtualBlob_MainBoard_0.4.0\uid__4-130^DesignRootModel_PCB_ESP32-C3-MINI-1_V1(2)_PCB_ESP32.ipt
- C:\Users\micyg\Projects\virtual_pet\VirtualBlob\Mechanical\boards\MainBoard\MainBoard_0_4_0\VirtualBlob_MainBoard_0.4.0\VirtualBlob_MainBoard_0.4.0\uid__4-131^DesignRootModel_PCB_ESP32-C3-MINI-1_V1(2)_PCB_ESP32.ipt
- C:\Users\micyg\Projects\virtual_pet\VirtualBlob\Mechanical\boards\MainBoard\MainBoard_0_4_0\VirtualBlob_MainBoard_0.4.0\VirtualBlob_MainBoard_0.4.0\uid__4-132^DesignRootModel_PCB_ESP32-C3-MINI-1_V1(2)_PCB_ESP32.ipt
- C:\Users\micyg\Projects\virtual_pet\VirtualBlob\Mechanical\boards\MainBoard\MainBoard_0_4_0\VirtualBlob_MainBoard_0.4.0\VirtualBlob_MainBoard_0.4.0\uid__4-133^DesignRootModel_PCB_ESP32-C3-MINI-1_V1(2)_PCB_ESP32.ipt
- C:\Users\micyg\Projects\virtual_pet\VirtualBlob\Mechanical\boards\MainBoard\MainBoard_0_4_0\VirtualBlob_MainBoard_0.4.0\VirtualBlob_MainBoard_0.4.0\uid__4-134^DesignRootModel_PCB_ESP32-C3-MINI-1_V1(2)_PCB_ESP32.ipt
- C:\Users\micyg\Projects\virtual_pet\VirtualBlob\Mechanical\boards\MainBoard\MainBoard_0_4_0\VirtualBlob_MainBoard_0.4.0\VirtualBlob_MainBoard_0.4.0\uid__4-135^DesignRootModel_PCB_ESP32-C3-MINI-1_V1(2)_PCB_ESP32.ipt
- C:\Users\micyg\Projects\virtual_pet\VirtualBlob\Mechanical\boards\MainBoard\MainBoard_0_4_0\VirtualBlob_MainBoard_0.4.0\VirtualBlob_MainBoard_0.4.0\uid__4-136^DesignRootModel_PCB_ESP32-C3-MINI-1_V1(2)_PCB_ESP32.ipt
- C:\Users\micyg\Projects\virtual_pet\VirtualBlob\Mechanical\boards\MainBoard\MainBoard_0_4_0\VirtualBlob_MainBoard_0.4.0\VirtualBlob_MainBoard_0.4.0\uid__4-137^DesignRootModel_PCB_ESP32-C3-MINI-1_V1(2)_PCB_ESP32.ipt
- C:\Users\micyg\Projects\virtual_pet\VirtualBlob\Mechanical\boards\MainBoard\MainBoard_0_4_0\VirtualBlob_MainBoard_0.4.0\VirtualBlob_MainBoard_0.4.0\uid__4-138^DesignRootModel_PCB_ESP32-C3-MINI-1_V1(2)_PCB_ESP32.ipt
- C:\Users\micyg\Projects\virtual_pet\VirtualBlob\Mechanical\boards\MainBoard\MainBoard_0_4_0\VirtualBlob_MainBoard_0.4.0\VirtualBlob_MainBoard_0.4.0\uid__4-139^DesignRootModel_PCB_ESP32-C3-MINI-1_V1(2)_PCB_ESP32.ipt
- C:\Users\micyg\Projects\virtual_pet\VirtualBlob\Mechanical\boards\MainBoard\MainBoard_0_4_0\VirtualBlob_MainBoard_0.4.0\VirtualBlob_MainBoard_0.4.0\uid__4-140^DesignRootModel_PCB_ESP32-C3-MINI-1_V1(2)_PCB_ESP32.ipt
- C:\Users\micyg\Projects\virtual_pet\VirtualBlob\Mechanical\boards\MainBoard\MainBoard_0_4_0\VirtualBlob_MainBoard_0.4.0\VirtualBlob_MainBoard_0.4.0\uid__4-141^DesignRootModel_PCB_ESP32-C3-MINI-1_V1(2)_PCB_ESP32.ipt
- C:\Users\micyg\Projects\virtual_pet\VirtualBlob\Mechanical\boards\MainBoard\MainBoard_0_4_0\VirtualBlob_MainBoard_0.4.0\VirtualBlob_MainBoard_0.4.0\uid__4-142^DesignRootModel_PCB_ESP32-C3-MINI-1_V1(2)_PCB_ESP32.ipt
- C:\Users\micyg\Projects\virtual_pet\VirtualBlob\Mechanical\boards\MainBoard\MainBoard_0_4_0\VirtualBlob_MainBoard_0.4.0\VirtualBlob_MainBoard_0.4.0\uid__4-143^DesignRootModel_PCB_ESP32-C3-MINI-1_V1(2)_PCB_ESP32.ipt
- C:\Users\micyg\Projects\virtual_pet\VirtualBlob\Mechanical\boards\MainBoard\MainBoard_0_4_0\VirtualBlob_MainBoard_0.4.0\VirtualBlob_MainBoard_0.4.0\uid__4-144^DesignRootModel_PCB_ESP32-C3-MINI-1_V1(2)_PCB_ESP32.ipt
- C:\Users\micyg\Projects\virtual_pet\VirtualBlob\Mechanical\boards\MainBoard\MainBoard_0_4_0\VirtualBlob_MainBoard_0.4.0\VirtualBlob_MainBoard_0.4.0\uid__4-145^DesignRootModel_PCB_ESP32-C3-MINI-1_V1(2)_PCB_ESP32.ipt
- C:\Users\micyg\Projects\virtual_pet\VirtualBlob\Mechanical\boards\MainBoard\MainBoard_0_4_0\VirtualBlob_MainBoard_0.4.0\VirtualBlob_MainBoard_0.4.0\uid__4-146^DesignRootModel_PCB_ESP32-C3-MINI-1_V1(2)_PCB_ESP32.ipt
- C:\Users\micyg\Projects\virtual_pet\VirtualBlob\Mechanical\boards\MainBoard\MainBoard_0_4_0\VirtualBlob_MainBoard_0.4.0\VirtualBlob_MainBoard_0.4.0\uid__4-147^DesignRootModel_PCB_ESP32-C3-MINI-1_V1(2)_PCB_ESP32.ipt
- C:\Users\micyg\Projects\virtual_pet\VirtualBlob\Mechanical\boards\MainBoard\MainBoard_0_4_0\VirtualBlob_MainBoard_0.4.0\VirtualBlob_MainBoard_0.4.0\uid__4-148^DesignRootModel_PCB_ESP32-C3-MINI-1_V1(2)_PCB_ESP32.ipt
- C:\Users\micyg\Projects\virtual_pet\VirtualBlob\Mechanical\boards\MainBoard\MainBoard_0_4_0\VirtualBlob_MainBoard_0.4.0\VirtualBlob_MainBoard_0.4.0\uid__4-149^DesignRootModel_PCB_ESP32-C3-MINI-1_V1(2)_PCB_ESP32.ipt
- C:\Users\micyg\Projects\virtual_pet\VirtualBlob\Mechanical\boards\MainBoard\MainBoard_0_4_0\VirtualBlob_MainBoard_0.4.0\VirtualBlob_MainBoard_0.4.0\uid__4-150^DesignRootModel_PCB_ESP32-C3-MINI-1_V1(2)_PCB_ESP32.ipt
- C:\Users\micyg\Projects\virtual_pet\VirtualBlob\Mechanical\boards\MainBoard\MainBoard_0_4_0\VirtualBlob_MainBoard_0.4.0\VirtualBlob_MainBoard_0.4.0\uid__4-151^DesignRootModel_PCB_ESP32-C3-MINI-1_V1(2)_PCB_ESP32.ipt
- C:\Users\micyg\Projects\virtual_pet\VirtualBlob\Mechanical\boards\MainBoard\MainBoard_0_4_0\VirtualBlob_MainBoard_0.4.0\VirtualBlob_MainBoard_0.4.0\uid__4-152^DesignRootModel_PCB_ESP32-C3-MINI-1_V1(2)_PCB_ESP32.ipt
- C:\Users\micyg\Projects\virtual_pet\VirtualBlob\Mechanical\boards\MainBoard\MainBoard_0_4_0\VirtualBlob_MainBoard_0.4.0\VirtualBlob_MainBoard_0.4.0\uid__4-153^DesignRootModel_PCB_ESP32-C3-MINI-1_V1(2)_PCB_ESP32.ipt
- C:\Users\micyg\Projects\virtual_pet\VirtualBlob\Mechanical\boards\MainBoard\MainBoard_0_4_0\VirtualBlob_MainBoard_0.4.0\VirtualBlob_MainBoard_0.4.0\uid__4-154^DesignRootModel_PCB_ESP32-C3-MINI-1_V1(2)_PCB_ESP32.ipt
- C:\Users\micyg\Projects\virtual_pet\VirtualBlob\Mechanical\boards\MainBoard\MainBoard_0_4_0\VirtualBlob_MainBoard_0.4.0\VirtualBlob_MainBoard_0.4.0\uid__4-155^DesignRootModel_PCB_ESP32-C3-MINI-1_V1(2)_PCB_ESP32.ipt
- C:\Users\micyg\Projects\virtual_pet\VirtualBlob\Mechanical\boards\MainBoard\MainBoard_0_4_0\VirtualBlob_MainBoard_0.4.0\VirtualBlob_MainBoard_0.4.0\uid__4-156^DesignRootModel_PCB_ESP32-C3-MINI-1_V1(2)_PCB_ESP32.ipt
- C:\Users\micyg\Projects\virtual_pet\VirtualBlob\Mechanical\boards\MainBoard\MainBoard_0_4_0\VirtualBlob_MainBoard_0.4.0\VirtualBlob_MainBoard_0.4.0\uid__4-157^DesignRootModel_PCB_ESP32-C3-MINI-1_V1(2)_PCB_ESP32.ipt
- C:\Users\micyg\Projects\virtual_pet\VirtualBlob\Mechanical\boards\MainBoard\MainBoard_0_4_0\VirtualBlob_MainBoard_0.4.0\VirtualBlob_MainBoard_0.4.0\uid__4-158^DesignRootModel_PCB_ESP32-C3-MINI-1_V1(2)_PCB_ESP32.ipt
- C:\Users\micyg\Projects\virtual_pet\VirtualBlob\Mechanical\boards\MainBoard\MainBoard_0_4_0\VirtualBlob_MainBoard_0.4.0\VirtualBlob_MainBoard_0.4.0\uid__4-159^DesignRootModel_PCB_ESP32-C3-MINI-1_V1(2)_PCB_ESP32.ipt
- C:\Users\micyg\Projects\virtual_pet\VirtualBlob\Mechanical\boards\MainBoard\MainBoard_0_4_0\VirtualBlob_MainBoard_0.4.0\VirtualBlob_MainBoard_0.4.0\uid__4-160^DesignRootModel_PCB_ESP32-C3-MINI-1_V1(2)_PCB_ESP32.ipt
- C:\Users\micyg\Projects\virtual_pet\VirtualBlob\Mechanical\boards\MainBoard\MainBoard_0_4_0\VirtualBlob_MainBoard_0.4.0\VirtualBlob_MainBoard_0.4.0\uid__1^DesignRootModel_PCB_ESP32-C3-MINI-1_V1(2)_PCB_ESP32-C3-.ipt
- C:\Users\micyg\Projects\virtual_pet\VirtualBlob\Mechanical\boards\MainBoard\MainBoard_0_4_0\VirtualBlob_MainBoard_0.4.0\VirtualBlob_MainBoard_0.4.0\uid__1-161^DesignRootModel_PCB_ESP32-C3-MINI-1_V1(2)_PCB_ESP32.ipt
- C:\Users\micyg\Projects\virtual_pet\VirtualBlob\Mechanical\boards\MainBoard\MainBoard_0_4_0\VirtualBlob_MainBoard_0.4.0\VirtualBlob_MainBoard_0.4.0\uid__1-162^DesignRootModel_PCB_ESP32-C3-MINI-1_V1(2)_PCB_ESP32.ipt
- C:\Users\micyg\Projects\virtual_pet\VirtualBlob\Mechanical\boards\MainBoard\MainBoard_0_4_0\VirtualBlob_MainBoard_0.4.0\VirtualBlob_MainBoard_0.4.0\uid__1-163^DesignRootModel_PCB_ESP32-C3-MINI-1_V1(2)_PCB_ESP32.ipt
- C:\Users\micyg\Projects\virtual_pet\VirtualBlob\Mechanical\boards\MainBoard\MainBoard_0_4_0\VirtualBlob_MainBoard_0.4.0\VirtualBlob_MainBoard_0.4.0\uid__1-164^DesignRootModel_PCB_ESP32-C3-MINI-1_V1(2)_PCB_ESP32.ipt
- C:\Users\micyg\Projects\virtual_pet\VirtualBlob\Mechanical\boards\MainBoard\MainBoard_0_4_0\VirtualBlob_MainBoard_0.4.0\VirtualBlob_MainBoard_0.4.0\uid__1-165^DesignRootModel_PCB_ESP32-C3-MINI-1_V1(2)_PCB_ESP32.ipt
- C:\Users\micyg\Projects\virtual_pet\VirtualBlob\Mechanical\boards\MainBoard\MainBoard_0_4_0\VirtualBlob_MainBoard_0.4.0\VirtualBlob_MainBoard_0.4.0\uid__1-166^DesignRootModel_PCB_ESP32-C3-MINI-1_V1(2)_PCB_ESP32.ipt
- C:\Users\micyg\Projects\virtual_pet\VirtualBlob\Mechanical\boards\MainBoard\MainBoard_0_4_0\VirtualBlob_MainBoard_0.4.0\VirtualBlob_MainBoard_0.4.0\uid__1-167^DesignRootModel_PCB_ESP32-C3-MINI-1_V1(2)_PCB_ESP32.ipt
- C:\Users\micyg\Projects\virtual_pet\VirtualBlob\Mechanical\boards\MainBoard\MainBoard_0_4_0\VirtualBlob_MainBoard_0.4.0\VirtualBlob_MainBoard_0.4.0\uid__1-168^DesignRootModel_PCB_ESP32-C3-MINI-1_V1(2)_PCB_ESP32.ipt